# Autodesk Inventor assembly: Shoulder+servo
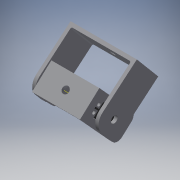
[picture p0: Inventor's stored thumbnail of the model, 180x180]
Saved by Autodesk Inventor 2018 (Build 220112000, 112)
## iProperties
Created: 2018-02-09
Part Number: Shoulder+servo
Material: Générique
Document SubType Name: Assembly
Designer: Thomas
Author: Thomas
## Documents named in this file (4)
- D:\Users\Thomas\Desktop\Projet robot augmenté\robotConcept\Shoulder\Shoulder+servo.iam
- D:\Users\Thomas\Desktop\Projet robot augmenté\robotConcept\MG996R SERVO\MG_996R.iam
- D:\Users\Thomas\Desktop\Projet robot augmenté\robotConcept\Shoulder\ShoulderPart1.ipt
- D:\Users\Thomas\Desktop\Projet robot augmenté\robotConcept\Shoulder\ShoulderPart2.ipt
## Components (3 placed, 3 different names)
1. MG_996R:1 [sub-assembly] — Placage:1, Rotation:1, Rotation:2, Placage:2, Rotation:3
2. ShoulderPart1:1 — Placage:1, Rotation:1, Rotation:2
3. ShoulderPart2:1 — Placage:2, Rotation:3
## Relationships (5: RevoluteJoint 3, Mate 2)
- Placage:1 [Mate]: MG_996R:1 ↔ ShoulderPart1:1
- Rotation:1 [RevoluteJoint]: MG_996R:1 ↔ ShoulderPart1:1
- Rotation:2 [RevoluteJoint]: MG_996R:1 ↔ ShoulderPart1:1
- Placage:2 [Mate]: MG_996R:1 ↔ ShoulderPart2:1
- Rotation:3 [RevoluteJoint]: MG_996R:1 ↔ ShoulderPart2:1
